# Autodesk Inventor assembly: F1.0256
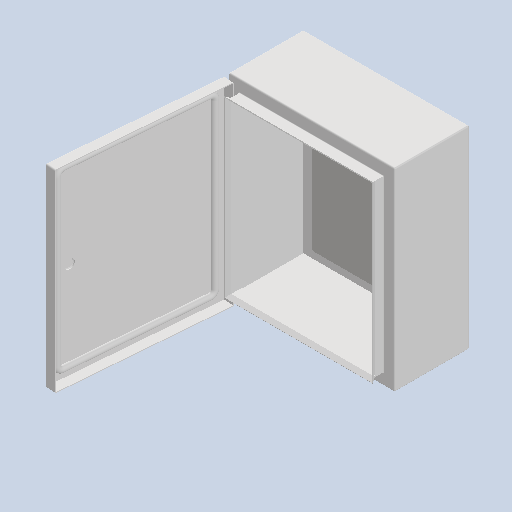
[picture p0: Inventor's stored thumbnail of the model, 512x512]
Saved by Autodesk Inventor 2022 (Build 260153000, 153)
## iProperties
Created: 2024-10-27
Part Number: F1.0256
Document SubType Name: Assembly
Designer: NANOmatic
Author: NANOmatic
## Documents named in this file (4)
- C:\Users\NANOmatic\Downloads\TomaszGwizdak\3D\F1.0256\F1.0256.iam
- C:\Users\NANOmatic\Downloads\TomaszGwizdak\3D\F1.0256\Sheet.ipt
- C:\Users\NANOmatic\Downloads\TomaszGwizdak\3D\F1.0256\Box.ipt
- C:\Users\NANOmatic\Downloads\TomaszGwizdak\3D\F1.0256\Door.ipt
## Components (3 placed, 3 different names)
1. Sheet:1 — Zestawiające:1, Równoległe:1, Równoległe:2
2. Box:1 — Zestawiające:1, Równoległe:1, Równoległe:2, Równoległe:3, Równoległe:4, Równoległe:5, Równoległe:6, Zestawiające:3, Zestawiające:4, Kątowe:1
3. Door:1 — Równoległe:6, Zestawiające:3, Zestawiające:4, Kątowe:1
## Relationships (10: Flush 6, Mate 3, Angle 1)
- Zestawiające:1 [Mate] (5 mm): Sheet:1 ↔ Box:1
- Równoległe:1 [Flush]: Sheet:1 ↔ Box:1
- Równoległe:2 [Flush]: Sheet:1 ↔ Box:1
- Równoległe:3 [Flush]: Box:1
- Równoległe:4 [Flush]: Box:1
- Równoległe:5 [Flush]: Box:1
- Równoległe:6 [Flush]: Box:1 ↔ Door:1
- Zestawiające:3 [Mate]: Box:1 ↔ Door:1
- Zestawiające:4 [Mate]: Box:1 ↔ Door:1
- Kątowe:1 [Angle] (0 deg): Box:1 ↔ Door:1
